# Autodesk Inventor assembly: LegLeftNCS
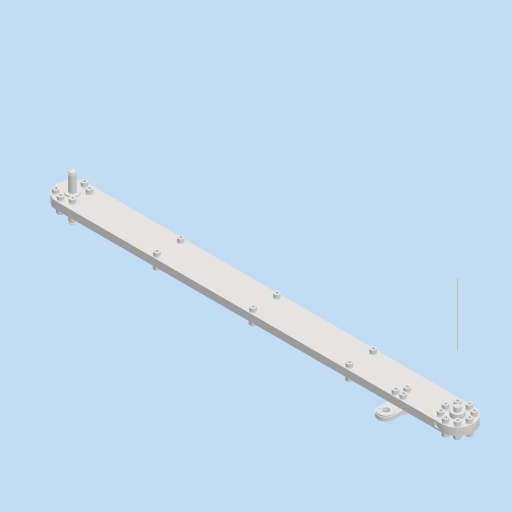
[picture p0: Inventor's stored thumbnail of the model, 512x512]
Saved by Autodesk Inventor 2023 (Build 270158000, 158)
## iProperties
Created: 2026-06-18
Part Number: LegLeftNCS
Document SubType Name: Assembly
Designer: Nathann
Author: Nathann
## Documents named in this file (2)
- C:\Users\Nathann\ClawdDrive\Objet3D\RunningRobot\PartURDF\LegLeftNCS.iam
- C:\Users\Nathann\ClawdDrive\Objet3D\RunningRobot\PartURDF\LegLeft.iam
## Components (1 placed, 1 different names)
1. LegLeft:1 [sub-assembly] — Mate:1, Flush:1, Flush:2, Flush:3, Flush:4
## Relationships (11: Mate 5, Flush 4, Symmetry 2)
- Mate:1: LegLeft:1
- Mate:2
- Mate:3
- Flush:1: LegLeft:1
- Flush:2: LegLeft:1
- Symmetry:1
- Mate:4
- Flush:3: LegLeft:1
- Flush:4: LegLeft:1
- Symmetry:2
- Mate:5
